# Autodesk Inventor assembly: ForearmActuatorBody
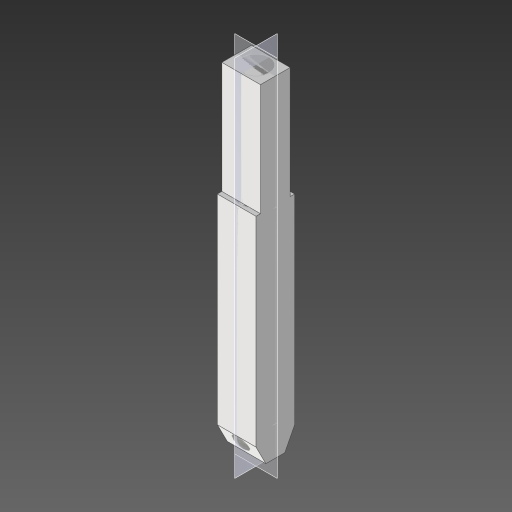
[picture p0: Inventor's stored thumbnail of the model, 512x512]
Saved by Autodesk Inventor 2023 (Build 270158000, 158)
## iProperties
Created: 2023-03-25
Part Number: ForearmActuatorBody
Document SubType Name: Assembly
Designer: Val
Author: Val
## Documents named in this file (3)
- C:\Users\Val\Desktop\str1ker\parts\external\ForearmActuator\ForearmActuatorBody.iam
- C:\Users\Val\Desktop\str1ker\parts\external\ForearmActuatorBody.ipt
- C:\Users\Val\Desktop\str1ker\description\models\src\ForearmActuatorBodyBoundingBox.ipt
## Components (2 placed, 2 different names)
1. ForearmActuatorBody:1 — Angle:1, Angle:2, Mate:1
2. ForearmActuatorBodyBoundingBox:1 — Flush:1
## Relationships (4: Angle 2, Mate 1, Flush 1)
- Angle:1 (180 deg): ForearmActuatorBody:1
- Angle:2 (180 deg): ForearmActuatorBody:1
- Mate:1: ForearmActuatorBody:1
- Flush:1: ForearmActuatorBodyBoundingBox:1
